# Autodesk Inventor assembly: Toughbox-mini with long shaft
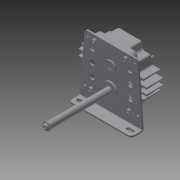
[picture p0: Inventor's stored thumbnail of the model, 180x180]
Saved by Autodesk Inventor 2014 SP1 (Build 180222100, 222)
## iProperties
Created: 2014-01-16
Part Number: Toughbox-mini with long shaft
Document SubType Name: Assembly
Designer: Pradhan Alexander
Author: Unknown
Title: S:/Products/Gearboxes Spur Single Stage/Toughbox/Toughbox Mini/Toughbox-Mini.stp
Organization: Unknown
Description: Unknown
Sending System: Unknown
Preprocessor: XStep 1.0
Author: Pradhan Alexander
## Documents named in this file (19)
- K:\MHS\Technology\Holliday B\Group Projects\Robotics\CAD Team\CAD Team 2014\Chassis 2014\Toughbox-mini with long shaft.iam
- K:\MHS\Technology\Holliday B\Group Projects\Robotics\CAD Team\CAD Team 2014\Chassis 2014\Imported Components\Toughbox-mini\r6zz.ipt
- K:\MHS\Technology\Holliday B\Group Projects\Robotics\CAD Team\CAD Team 2014\Chassis 2014\Imported Components\Toughbox-mini\Toughbox_d07.ipt
- K:\MHS\Technology\Holliday B\Group Projects\Robotics\CAD Team\CAD Team 2014\Chassis 2014\Imported Components\Toughbox-mini\Toughbox_d05.ipt
- K:\MHS\Technology\Holliday B\Group Projects\Robotics\CAD Team\CAD Team 2014\Chassis 2014\Imported Components\Toughbox-mini\Toughbox_d08.ipt
- K:\MHS\Technology\Holliday B\Group Projects\Robotics\CAD Team\CAD Team 2014\Chassis 2014\Imported Components\Toughbox-mini\Toughbox_d06.ipt
- K:\MHS\Technology\Holliday B\Group Projects\Robotics\CAD Team\CAD Team 2014\Chassis 2014\Imported Components\Toughbox-mini\fr-6-zz.ipt
- K:\MHS\Technology\Holliday B\Group Projects\Robotics\CAD Team\CAD Team 2014\Chassis 2014\Imported Components\Toughbox-mini\fr-8-zz.ipt
- K:\MHS\Technology\Holliday B\Group Projects\Robotics\CAD Team\CAD Team 2014\Chassis 2014\Imported Components\Toughbox-mini\10-32_nylock_nut.ipt
- K:\MHS\Technology\Holliday B\Group Projects\Robotics\CAD Team\CAD Team 2014\Chassis 2014\Imported Components\Toughbox-mini\5-16_washer.ipt
- K:\MHS\Technology\Holliday B\Group Projects\Robotics\CAD Team\CAD Team 2014\Chassis 2014\Imported Components\Toughbox-mini\Toughbox_d09.ipt
- K:\MHS\Technology\Holliday B\Group Projects\Robotics\CAD Team\CAD Team 2014\Chassis 2014\Imported Components\Toughbox-mini\8mm_spring_clip.ipt
- K:\MHS\Technology\Holliday B\Group Projects\Robotics\CAD Team\CAD Team 2014\Chassis 2014\Imported Components\Toughbox-mini\Toughbox-mini_d01-5-12.ipt
- K:\MHS\Technology\Holliday B\Group Projects\Robotics\CAD Team\CAD Team 2014\Chassis 2014\Imported Components\Toughbox-mini\Toughbox-mini_d02.ipt
- K:\MHS\Technology\Holliday B\Group Projects\Robotics\CAD Team\CAD Team 2014\Chassis 2014\Imported Components\Toughbox-mini\250_washer.ipt
- K:\MHS\Technology\Holliday B\Group Projects\Robotics\CAD Team\CAD Team 2014\Chassis 2014\Imported Components\Toughbox-mini\14-20x0500_bhcs.ipt
- K:\MHS\Technology\Holliday B\Group Projects\Robotics\CAD Team\CAD Team 2014\Chassis 2014\Imported Components\Toughbox-mini\125x124x700_key.ipt
- K:\MHS\Technology\Holliday B\Group Projects\Robotics\CAD Team\CAD Team 2014\Chassis 2014\Imported Components\Toughbox-mini\10-32x0625_shcs.ipt
- K:\MHS\Technology\Holliday B\Group Projects\Robotics\CAD Team\CAD Team 2014\Chassis 2014\Imported Components\Toughbox-d28\Toughbox-d28.ipt
## Components (34 placed, 18 different names)
1. r6zz
2. r6zz:1
3. Toughbox_d07
4. Toughbox_d05
5. Toughbox_d08
6. Toughbox_d06
7. fr-6-zz
8. fr-8-zz — Insert:1
9. 10-32_nylock_nut
10. 10-32_nylock_nut:1
11. 10-32_nylock_nut:2
12. 10-32_nylock_nut:3
13. 5-16_washer
14. 5-16_washer:1
15. 5-16_washer:2
16. 5-16_washer:3
17. Toughbox_d09
18. Toughbox_d09:1
19. 8mm_spring_clip
20. 8mm_spring_clip:1
21. Toughbox-mini_d01-5-12 — Insert:4, Insert:5
22. Toughbox-mini_d02 — Insert:4, Insert:5
23. 250_washer — Insert:2, Insert:3
24. 14-20x0500_bhcs — Insert:3
25. 125x124x700_key — Mate:1, Mate:2
26. 10-32x0625_shcs
27. 10-32x0625_shcs:1
28. 10-32x0625_shcs:2
29. 10-32x0625_shcs:3
30. 10-32x0625_shcs:4
31. 10-32x0625_shcs:5
32. 10-32x0625_shcs:6
33. 10-32x0625_shcs:7
34. Toughbox-d28:1 — Insert:1, Insert:2, Mate:1, Mate:2
## Relationships (7: Insert 5, Mate 2)
- Insert:1: fr-8-zz ↔ Toughbox-d28:1
- Insert:2: 250_washer ↔ Toughbox-d28:1
- Insert:3: 250_washer ↔ 14-20x0500_bhcs
- Mate:1: 125x124x700_key ↔ Toughbox-d28:1
- Mate:2: 125x124x700_key ↔ Toughbox-d28:1
- Insert:4: Toughbox-mini_d01-5-12 ↔ Toughbox-mini_d02
- Insert:5: Toughbox-mini_d01-5-12 ↔ Toughbox-mini_d02
